# Autodesk Inventor assembly: Shoulder base
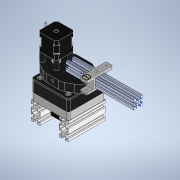
[picture p0: Inventor's stored thumbnail of the model, 180x180]
Saved by Autodesk Inventor 2022 (Build 260153000, 153)
## iProperties
Created: 2022-03-02
Part Number: Shoulder base
Document SubType Name: Assembly
Designer: JK
Author: JK
## Documents named in this file (19)
- C:\Users\JK\Documents\Inventor\ScaraNema\SCARA-3DP\Parts\Shoulder\Shoulder base.iam
- C:\Users\JK\Documents\Inventor\ScaraNema\SCARA-3DP\Parts\Shoulder\17HS15-1684S-PG5.ipt
- C:\Users\JK\Documents\Inventor\ScaraNema\SCARA-3DP\Parts\Shoulder\Motor Support Plate.ipt
- C:\Users\JK\Documents\Inventor\ScaraNema\SCARA-3DP\Parts\Shoulder\Base.ipt
- C:\Users\JK\Documents\Inventor\ScaraNema\SCARA-3DP\Parts\Shoulder\Needle roller bearing\5909K79_1 mm Thick Washer for 45 mm Shaft Diameter Needle-Roller Thrust Bearing.ipt
- C:\Users\JK\Documents\Inventor\ScaraNema\SCARA-3DP\Parts\Shoulder\Needle roller bearing\5909K19_Needle-Roller Thrust Bearing.ipt
- C:\Users\JK\Documents\Inventor\ScaraNema\SCARA-3DP\Parts\Shoulder\ExtraBase.ipt
- C:\Users\JK\Documents\Inventor\ScaraNema\SCARA-3DP\Parts\Shoulder\V-Slot 20x40x83.ipt
- C:\Users\JK\Documents\Inventor\ScaraNema\SCARA-3DP\Parts\Shoulder\M5x45 flathead.ipt
- C:\Users\JK\Documents\Inventor\ScaraNema\SCARA-3DP\Parts\TuercaTM5Perfil2020.ipt
- C:\Users\JK\Documents\Inventor\ScaraNema\SCARA-3DP\Parts\Shoulder\Platform.ipt
- C:\Users\JK\Documents\Inventor\ScaraNema\SCARA-3DP\Parts\Shoulder\M3x6 sinkbolt.ipt
- C:\Users\JK\Documents\Inventor\ScaraNema\SCARA-3DP\Parts\Shoulder\Motor spacer.ipt
- C:\Users\JK\Documents\Inventor\ScaraNema\SCARA-3DP\Parts\Shoulder\MOTOR.ipt
- C:\Users\JK\Documents\Inventor\ScaraNema\SCARA-3DP\Parts\Shoulder\M3x35.ipt
- C:\Users\JK\Documents\Inventor\ScaraNema\SCARA-3DP\Parts\Shoulder\GT2 16 Pulley.ipt
- C:\Users\JK\Documents\Inventor\ScaraNema\SCARA-3DP\Parts\V-Slot 20x20\V-Slot 20x20x150.ipt
- C:\Users\JK\Documents\Inventor\ScaraNema\SCARA-3DP\Parts\V-Slot 20x20.ipt
- C:\Users\JK\Documents\Inventor\ScaraNema\SCARA-3DP\Parts\Shoulder\Belt tensor.ipt
## Components (34 placed, 17 different names)
1. 17HS15-1684S-PG5:1 — Coincidencia:1, Coincidencia:2, Coincidencia:3, Coincidencia:4, Coincidencia:9, Coincidencia:10, Coincidencia:22
2. Motor Support Plate:1 — Coincidencia:1, Coincidencia:2, Coincidencia:3, Coincidencia:5, Coincidencia:6, Coincidencia:7, Coincidencia:8, Coincidencia:13, Coincidencia:14, Coincidencia:18, Coincidencia:19, Coincidencia:24, Nivelación:6
3. Base:1 — Coincidencia:4, Coincidencia:5, Coincidencia:6, Coincidencia:15, Nivelación:2
4. 5909K79_1 mm Thick Washer for 45 mm Shaft Diameter Needle-Roller Thrust Bearing:1 — Coincidencia:7, Coincidencia:8, Tangente:1
5. 5909K19_Needle-Roller Thrust Bearing:1 — Coincidencia:9, Tangente:1, Tangente:2
6. 5909K79_1 mm Thick Washer for 45 mm Shaft Diameter Needle-Roller Thrust Bearing:2 — Coincidencia:10, Tangente:2, Coincidencia:23
7. ExtraBase:1 — Coincidencia:13, Coincidencia:14, Coincidencia:15, Coincidencia:16, Coincidencia:17, Nivelación:3, Nivelación:4, Nivelación:5
8. V-Slot 20x40x83:1 — Coincidencia:17, Nivelación:1, Nivelación:3, Nivelación:4
9. V-Slot 20x40x83:2 — Coincidencia:16, Nivelación:1, Nivelación:2, Nivelación:5, Ángulo:1, Coincidencia:21
10. Platform:1 — Coincidencia:22, Coincidencia:23, Coincidencia:25, Coincidencia:26, Coincidencia:30, Nivelación:7, Ángulo:2, Coincidencia:32, Coincidencia:33, Nivelación:8
11. MOTOR:1 — Coincidencia:28, Coincidencia:31, Ángulo:2, Coincidencia:32, Coincidencia:34
12. GT2 16 Pulley:1 — Coincidencia:31, Nivelación:7
13. V-Slot 20x20x150:1 — Coincidencia:33, Nivelación:8, Coincidencia:34, Coincidencia:35, Coincidencia:36, Nivelación:9
14. Belt tensor:1 — Coincidencia:35, Coincidencia:36, Nivelación:9
15. M5x45 flathead:1 — Coincidencia:18, Coincidencia:19, Coincidencia:20
16. TuercaTM5Perfil2020:1 — Coincidencia:20, Ángulo:1, Coincidencia:21
17. M5x45 flathead:2
18. TuercaTM5Perfil2020:2
19. M5x45 flathead:3
20. TuercaTM5Perfil2020:3
21. M5x45 flathead:4
22. TuercaTM5Perfil2020:4
23. M3x6 sinkbolt:1 — Coincidencia:24, Nivelación:6
24. M3x6 sinkbolt:2
25. M3x6 sinkbolt:3
26. M3x6 sinkbolt:4
27. M3x35:1 — Coincidencia:29, Coincidencia:30
28. Motor spacer:1 — Coincidencia:25, Coincidencia:26, Coincidencia:28, Coincidencia:29
29. M3x35:2
30. Motor spacer:2
31. M3x35:3
32. Motor spacer:3
33. M3x35:4
34. Motor spacer:4
## Component patterns: (4 elements, first: M5x45 flathead:1 + TuercaTM5Perfil2020:1), (4 elements, first: M3x6 sinkbolt:1), (4 elements, first: M3x35:1 + Motor spacer:1)
## Relationships (46: Mate 33, Flush 9, Tangent 2, Angle 2)
- Coincidencia:1 [Mate]: 17HS15-1684S-PG5:1 ↔ Motor Support Plate:1
- Coincidencia:2 [Mate]: 17HS15-1684S-PG5:1 ↔ Motor Support Plate:1
- Coincidencia:3 [Mate]: 17HS15-1684S-PG5:1 ↔ Motor Support Plate:1
- Coincidencia:4 [Mate]: 17HS15-1684S-PG5:1 ↔ Base:1
- Coincidencia:5 [Mate]: Motor Support Plate:1 ↔ Base:1
- Coincidencia:6 [Mate]: Motor Support Plate:1 ↔ Base:1
- Coincidencia:7 [Mate]: Motor Support Plate:1 ↔ 5909K79_1 mm Thick Washer for 45 mm Shaft Diameter Needle-Roller Thrust Bearing:1
- Coincidencia:8 [Mate]: Motor Support Plate:1 ↔ 5909K79_1 mm Thick Washer for 45 mm Shaft Diameter Needle-Roller Thrust Bearing:1
- Coincidencia:9 [Mate]: 17HS15-1684S-PG5:1 ↔ 5909K19_Needle-Roller Thrust Bearing:1
- Tangente:1: 5909K79_1 mm Thick Washer for 45 mm Shaft Diameter Needle-Roller Thrust Bearing:1 ↔ 5909K19_Needle-Roller Thrust Bearing:1
- Coincidencia:10 [Mate]: 17HS15-1684S-PG5:1 ↔ 5909K79_1 mm Thick Washer for 45 mm Shaft Diameter Needle-Roller Thrust Bearing:2
- Tangente:2: 5909K19_Needle-Roller Thrust Bearing:1 ↔ 5909K79_1 mm Thick Washer for 45 mm Shaft Diameter Needle-Roller Thrust Bearing:2
- Coincidencia:13 [Mate]: Motor Support Plate:1 ↔ ExtraBase:1
- Coincidencia:14 [Mate]: Motor Support Plate:1 ↔ ExtraBase:1
- Coincidencia:15 [Mate]: Base:1 ↔ ExtraBase:1
- Coincidencia:16 [Mate]: ExtraBase:1 ↔ V-Slot 20x40x83:2
- Coincidencia:17 [Mate]: ExtraBase:1 ↔ V-Slot 20x40x83:1
- Nivelación:1 [Flush]: V-Slot 20x40x83:1 ↔ V-Slot 20x40x83:2
- Nivelación:2 [Flush]: Base:1 ↔ V-Slot 20x40x83:2
- Nivelación:3 [Flush]: ExtraBase:1 ↔ V-Slot 20x40x83:1
- Nivelación:4 [Flush] (-0.35 mm): ExtraBase:1 ↔ V-Slot 20x40x83:1
- Nivelación:5 [Flush]: ExtraBase:1 ↔ V-Slot 20x40x83:2
- Coincidencia:18 [Mate]: Motor Support Plate:1 ↔ M5x45 flathead:1
- Coincidencia:19 [Mate]: Motor Support Plate:1 ↔ M5x45 flathead:1
- Coincidencia:20 [Mate]: M5x45 flathead:1 ↔ TuercaTM5Perfil2020:1
- Ángulo:1 [Angle] (0 deg): V-Slot 20x40x83:2 ↔ TuercaTM5Perfil2020:1
- Coincidencia:21 [Mate] (1.15 mm): V-Slot 20x40x83:2 ↔ TuercaTM5Perfil2020:1
- Coincidencia:22 [Mate]: 17HS15-1684S-PG5:1 ↔ Platform:1
- Coincidencia:23 [Mate]: 5909K79_1 mm Thick Washer for 45 mm Shaft Diameter Needle-Roller Thrust Bearing:2 ↔ Platform:1
- Coincidencia:24 [Mate]: Motor Support Plate:1 ↔ M3x6 sinkbolt:1
- Nivelación:6 [Flush]: Motor Support Plate:1 ↔ M3x6 sinkbolt:1
- Coincidencia:25 [Mate]: Platform:1 ↔ Motor spacer:1
- Coincidencia:26 [Mate]: Platform:1 ↔ Motor spacer:1
- Coincidencia:28 [Mate]: MOTOR:1 ↔ Motor spacer:1
- Coincidencia:29 [Mate]: M3x35:1 ↔ Motor spacer:1
- Coincidencia:30 [Mate]: Platform:1 ↔ M3x35:1
- Coincidencia:31 [Mate]: MOTOR:1 ↔ GT2 16 Pulley:1
- Nivelación:7 [Flush] (-6.25 mm): Platform:1 ↔ GT2 16 Pulley:1
- Ángulo:2 [Angle] (90 deg): Platform:1 ↔ MOTOR:1
- Coincidencia:32 [Mate]: Platform:1 ↔ MOTOR:1
- Coincidencia:33 [Mate]: Platform:1 ↔ V-Slot 20x20x150:1
- Nivelación:8 [Flush] (-25 mm): Platform:1 ↔ V-Slot 20x20x150:1
- Coincidencia:34 [Mate] (10 mm): MOTOR:1 ↔ V-Slot 20x20x150:1
- Coincidencia:35 [Mate] (0.15 mm): V-Slot 20x20x150:1 ↔ Belt tensor:1
- Coincidencia:36 [Mate] (0.15 mm): V-Slot 20x20x150:1 ↔ Belt tensor:1
- Nivelación:9 [Flush] (-50 mm): V-Slot 20x20x150:1 ↔ Belt tensor:1
